# Autodesk Inventor assembly: First Technolgical stage Table Top Assembly
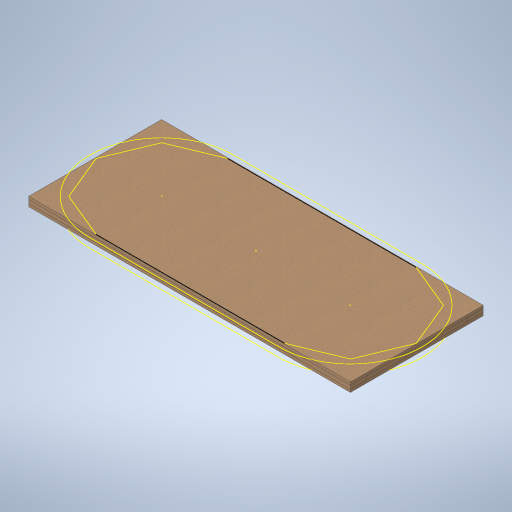
[picture p0: Inventor's stored thumbnail of the model, 512x512]
Saved by Autodesk Inventor 2024 (Build 280153000, 153)
## iProperties
Created: 2020-04-16
Part Number: First Technolgical stage Table Top Assembly
Document SubType Name: Assembly
Designer: SauliusD
Author: SauliusD
## Documents named in this file (6)
- C:\W4INV 2024 Design\PROJECTS\Samples\Composite Material Table\1 Technolgical stage\First Technolgical stage Table Top Assembly.iam
- C:\W4INV 2024 Design\PROJECTS\Samples\Composite Material Table\1 Technolgical stage\Side Insert plank.ipt
- C:\W4INV 2024 Design\PROJECTS\Samples\Composite Material Table\1 Technolgical stage\Cover Board.ipt
- C:\W4INV 2024 Design\PROJECTS\Samples\Composite Material Table\1 Technolgical stage\Between Side Insert.ipt
- C:\W4INV 2024 Design\PROJECTS\Samples\Composite Material Table\1 Technolgical stage\Between Inner Insert.ipt
- C:\W4INV 2024 Design\PROJECTS\Samples\Composite Material Table\Composite Top Table Skeleton.ipt
## Components (9 placed, 4 different names)
1. Side Insert plank:1 — Mate:2, Mate:5
2. Cover Board:1 — Mate:1, Mate:3
3. Between Side Insert:1
4. Between Side Insert:2 — Mate:1, Mate:2, Mate:4, Mate:6
5. Side Insert plank:2 — Mate:3, Mate:4
6. Cover Board:2 — Mate:5, Mate:6
7. Between Inner Insert:1
8. Between Inner Insert:2
9. Between Inner Insert:3
## Component patterns: (3 elements, first: Between Inner Insert:1)
## Relationships (6: Mate 6)
- Mate:1: Cover Board:1 ↔ Between Side Insert:2
- Mate:2: Side Insert plank:1 ↔ Between Side Insert:2
- Mate:3: Cover Board:1 ↔ Side Insert plank:2
- Mate:4: Between Side Insert:2 ↔ Side Insert plank:2
- Mate:5: Side Insert plank:1 ↔ Cover Board:2
- Mate:6: Between Side Insert:2 ↔ Cover Board:2
## Named parameters: BetweenInserts = 332.5 mm, InsertN = 3
